# Autodesk Inventor assembly: Inner
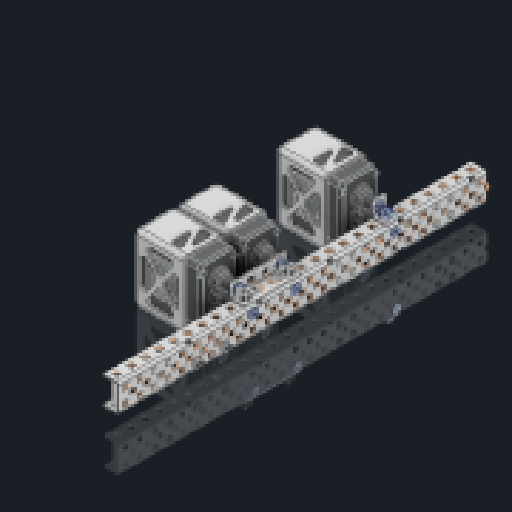
[picture p0: Inventor's stored thumbnail of the model, 512x512]
Saved by Autodesk Inventor 2025 (Build 290162000, 162)
## iProperties
Created: 2025-01-28
Part Number: Inner
Document SubType Name: Assembly
Designer: Averey Ku
Author: Averey Ku
## Documents named in this file (25)
- D:\VEX\High Stakes\CAD\V5\Chassis\Drivebay Left\Inner.iam
- D:\VEX\High Stakes\CAD\ROBOPROS-CAD-Inventor\Structure\C Channel\Aluminum 1x2x1\Alu C 1x2x1x26.ipt
- D:\VEX\High Stakes\CAD\ROBOPROS-CAD-Inventor\Structure\C Channel\Aluminum 1x3x1 Half\Alu C Half 1x3x1x1.ipt
- D:\VEX\High Stakes\CAD\ROBOPROS-CAD-Inventor\Electronics\Motor with Cover.iam
- D:\VEX\High Stakes\CAD\ROBOPROS-CAD-Inventor\Structure\C Channel\Aluminum 1x3x1 Half\Alu C Half 1x3x1x4.ipt
- D:\VEX\High Stakes\CAD\ROBOPROS-CAD-Inventor\Motion\Spacers\Spacer Nylon .313 OD\NSpacer .313 OD x .500.ipt
- D:\VEX\High Stakes\CAD\ROBOPROS-CAD-Inventor\Motion\Spacers\Spacer Nylon .313 OD.ipt
- D:\VEX\High Stakes\CAD\ROBOPROS-CAD-Inventor\Motion\Spacers\Washer Steel\SWasher .375 OD x .062500.ipt
- D:\VEX\High Stakes\CAD\ROBOPROS-CAD-Inventor\Motion\Spacers\Washer Steel.ipt
- D:\VEX\High Stakes\CAD\ROBOPROS-CAD-Inventor\Structure\Hardware\Screw Steel - Star\SScrew Star Smooth .250.ipt
- D:\VEX\High Stakes\CAD\ROBOPROS-CAD-Inventor\Structure\Hardware\Screw Steel - Star.ipt
- D:\VEX\High Stakes\CAD\ROBOPROS-CAD-Inventor\Structure\1-Post Standoff Retainer.ipt
- D:\VEX\High Stakes\CAD\ROBOPROS-CAD-Inventor\Structure\Standoff\Standoff .25.ipt
- D:\VEX\High Stakes\CAD\ROBOPROS-CAD-Inventor\Structure\Standoff.ipt
- D:\VEX\High Stakes\CAD\ROBOPROS-CAD-Inventor\Structure\Hardware\Screw Shoulder Robosource\SScrew Shoulder Smooth .500 x .04.ipt
- D:\VEX\High Stakes\CAD\ROBOPROS-CAD-Inventor\Structure\Hardware\Screw Shoulder Robosource.ipt
- D:\VEX\High Stakes\CAD\ROBOPROS-CAD-Inventor\Structure\Hardware\Screw Shoulder Robosource\SScrew Shoulder Smooth .375 x .12.ipt
- D:\VEX\High Stakes\CAD\ROBOPROS-CAD-Inventor\Structure\Hardware\Nut Nylock.ipt
- D:\VEX\High Stakes\CAD\ROBOPROS-CAD-Inventor\Structure\Hardware\Screw Steel - Star\SScrew Star Smooth .750.ipt
- D:\VEX\High Stakes\CAD\ROBOPROS-CAD-Inventor\Motion\Shaft LS\Bearing Flat Low Profile.ipt
- D:\VEX\High Stakes\CAD\ROBOPROS-CAD-Inventor\Structure\Hardware\Screw Nylon - Pan Head\NScrew Pan Head Threaded .500.ipt
- D:\VEX\High Stakes\CAD\ROBOPROS-CAD-Inventor\Structure\Hardware\Nut Nylon\Nut Nylon - White.ipt
- D:\VEX\High Stakes\CAD\ROBOPROS-CAD-Inventor\Structure\Hardware\Nut Nylon.ipt
- D:\VEX\High Stakes\CAD\ROBOPROS-CAD-Inventor\Structure\4-Post Hex Nut Retainer.ipt
- D:\VEX\High Stakes\CAD\ROBOPROS-CAD-Inventor\Structure\Nylon Standoff Rounded\Nylon Standoff .875.ipt
## Components (38 placed, 18 different names)
1. Alu C 1x2x1x26:1 — Insert:6, Mate:4, Insert:9, Insert:10, Insert:14, Insert:21, Insert:22, Insert:24, Insert:26, Insert:27, Insert:28, Insert:31, Insert:32, Insert:33, Mate:7, Insert:34, Mate:8, Insert:37, Mate:9, Insert:39, Mate:10, Insert:40
2. Alu C Half 1x3x1x1:1 — Insert:23, Insert:25
3. Motor with Cover:1 [sub-assembly] — Insert:7
4. Motor with Cover:2 [sub-assembly] — Insert:8
5. Motor with Cover:3 [sub-assembly]
6. Alu C Half 1x3x1x4:1 — Insert:6, Mate:4, Insert:7, Insert:8, Insert:15, Insert:16, Insert:17, Mate:5, Insert:18, Mate:6
7. NSpacer .313 OD x .500:1 — Insert:9, Insert:11
8. NSpacer .313 OD x .500:2 — Insert:10, Insert:12
9. SWasher .375 OD x .062500:1 — Insert:12
10. SWasher .375 OD x .062500:2 — Insert:11
11. NSpacer .313 OD x .500:3 — Insert:14
12. SWasher .375 OD x .062500:3
13. SScrew Star Smooth .250:1 — Insert:15
14. SScrew Star Smooth .250:2 — Insert:16
15. 1-Post Standoff Retainer:1 — Insert:17, Mate:5, Insert:19, Angle:1
16. 1-Post Standoff Retainer:2 — Insert:18, Mate:6, Insert:20, Angle:2
17. Standoff .25:1 — Insert:19, Angle:1
18. Standoff .25:2 — Insert:20, Angle:2
19. SScrew Shoulder Smooth .500 x .04:1 — Insert:22
20. SScrew Shoulder Smooth .500 x .04:2 — Insert:21
21. SScrew Star Smooth .250:3 — Insert:23
22. SScrew Shoulder Smooth .375 x .12:3 — Insert:24
23. Nut Nylock:1 — Insert:25
24. SScrew Star Smooth .750:4 — Insert:26
25. SScrew Star Smooth .750:5 — Insert:27
26. SScrew Star Smooth .750:6 — Insert:28
27. Bearing Flat Low Profile:1 — Insert:33, Mate:7
28. NScrew Pan Head Threaded .500:1 — Insert:31
29. Nut Nylon - White:1
30. Nut Nylon - White:2
31. NScrew Pan Head Threaded .500:2 — Insert:32
32. 4-Post Hex Nut Retainer:1 — Insert:34, Mate:8, Insert:35
33. Nut Nylock:2 — Insert:35
34. 4-Post Hex Nut Retainer:2 — Insert:37, Mate:9
35. Nut Nylock:3
36. 4-Post Hex Nut Retainer:3 — Insert:39, Mate:10
37. Nut Nylock:4
38. Nylon Standoff .875:1 — Insert:40
## Relationships (49: Insert 37, Mate 10, Angle 2)
- [Insert]: Alu C 1x2x1x26:1 ↔ Alu C Half 1x3x1x1:1
- [Mate]: Alu C 1x2x1x26:1 ↔ Motor with Cover:1
- [Mate]: Alu C 1x2x1x26:1 ↔ Motor with Cover:2
- [Insert]: Alu C Half 1x3x1x1:1 ↔ Motor with Cover:3
- [Mate]: Alu C 1x2x1x26:1 ↔ Motor with Cover:3
- Insert:6: Alu C 1x2x1x26:1 ↔ Alu C Half 1x3x1x4:1
- Mate:4: Alu C 1x2x1x26:1 ↔ Alu C Half 1x3x1x4:1
- Insert:7: Motor with Cover:1 ↔ Alu C Half 1x3x1x4:1
- Insert:8: Motor with Cover:2 ↔ Alu C Half 1x3x1x4:1
- Insert:9: Alu C 1x2x1x26:1 ↔ NSpacer .313 OD x .500:1
- Insert:10: Alu C 1x2x1x26:1 ↔ NSpacer .313 OD x .500:2
- Insert:11: NSpacer .313 OD x .500:1 ↔ SWasher .375 OD x .062500:2
- Insert:12: NSpacer .313 OD x .500:2 ↔ SWasher .375 OD x .062500:1
- [Insert]: NSpacer .313 OD x .500:3 ↔ SWasher .375 OD x .062500:3
- Insert:14: Alu C 1x2x1x26:1 ↔ NSpacer .313 OD x .500:3
- Insert:15: Alu C Half 1x3x1x4:1 ↔ SScrew Star Smooth .250:1
- Insert:16: Alu C Half 1x3x1x4:1 ↔ SScrew Star Smooth .250:2
- Insert:17: Alu C Half 1x3x1x4:1 ↔ 1-Post Standoff Retainer:1
- Mate:5: Alu C Half 1x3x1x4:1 ↔ 1-Post Standoff Retainer:1
- Insert:18: Alu C Half 1x3x1x4:1 ↔ 1-Post Standoff Retainer:2
- Mate:6: Alu C Half 1x3x1x4:1 ↔ 1-Post Standoff Retainer:2
- Insert:19: 1-Post Standoff Retainer:1 ↔ Standoff .25:1
- Angle:1 (0 deg): 1-Post Standoff Retainer:1 ↔ Standoff .25:1
- Insert:20: 1-Post Standoff Retainer:2 ↔ Standoff .25:2
- Angle:2 (0 deg): 1-Post Standoff Retainer:2 ↔ Standoff .25:2
- Insert:21: Alu C 1x2x1x26:1 ↔ SScrew Shoulder Smooth .500 x .04:2
- Insert:22: Alu C 1x2x1x26:1 ↔ SScrew Shoulder Smooth .500 x .04:1
- Insert:23: Alu C Half 1x3x1x1:1 ↔ SScrew Star Smooth .250:3
- Insert:24: Alu C 1x2x1x26:1 ↔ SScrew Shoulder Smooth .375 x .12:3
- Insert:25: Alu C Half 1x3x1x1:1 ↔ Nut Nylock:1
- Insert:26: Alu C 1x2x1x26:1 ↔ SScrew Star Smooth .750:4
- Insert:27: Alu C 1x2x1x26:1 ↔ SScrew Star Smooth .750:5
- Insert:28: Alu C 1x2x1x26:1 ↔ SScrew Star Smooth .750:6
- [Insert] (1.27 mm): Bearing Flat Low Profile:1 ↔ Nut Nylon - White:1
- [Insert] (1.27 mm): Bearing Flat Low Profile:1 ↔ Nut Nylon - White:2
- Insert:31: Alu C 1x2x1x26:1 ↔ NScrew Pan Head Threaded .500:1
- Insert:32: Alu C 1x2x1x26:1 ↔ NScrew Pan Head Threaded .500:2
- Insert:33: Alu C 1x2x1x26:1 ↔ Bearing Flat Low Profile:1
- Mate:7: Alu C 1x2x1x26:1 ↔ Bearing Flat Low Profile:1
- Insert:34: Alu C 1x2x1x26:1 ↔ 4-Post Hex Nut Retainer:1
- Mate:8: Alu C 1x2x1x26:1 ↔ 4-Post Hex Nut Retainer:1
- Insert:35: 4-Post Hex Nut Retainer:1 ↔ Nut Nylock:2
- [Insert]: 4-Post Hex Nut Retainer:2 ↔ Nut Nylock:3
- Insert:37: Alu C 1x2x1x26:1 ↔ 4-Post Hex Nut Retainer:2
- Mate:9: Alu C 1x2x1x26:1 ↔ 4-Post Hex Nut Retainer:2
- [Insert]: 4-Post Hex Nut Retainer:3 ↔ Nut Nylock:4
- Insert:39: Alu C 1x2x1x26:1 ↔ 4-Post Hex Nut Retainer:3
- Mate:10: Alu C 1x2x1x26:1 ↔ 4-Post Hex Nut Retainer:3
- Insert:40: Alu C 1x2x1x26:1 ↔ Nylon Standoff .875:1
## Named parameters: d18_d17 = 0 mm, d52_d51 = 0 mm, d55_d51 = 0 mm
